# Autodesk Inventor assembly: Ensamble Atril
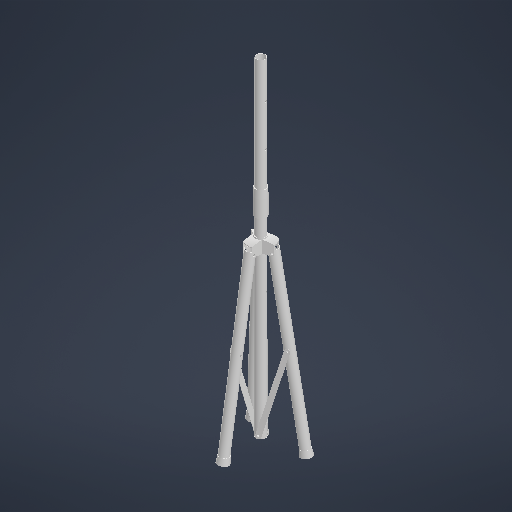
[picture p0: Inventor's stored thumbnail of the model, 512x512]
Saved by Autodesk Inventor 2026.2 (Build 302298000, 298)
## iProperties
Created: 2026-01-05
Part Number: Ensamble Atril
Document SubType Name: Assembly
Designer: vicho
Author: vicho
## Documents named in this file (8)
- C:\Users\vicho\OneDrive\Documentos\PROYECTOS INVENTOR\atril\Ensamble Atril.iam
- C:\Users\vicho\OneDrive\Documentos\PROYECTOS INVENTOR\atril\Pieza37.ipt
- C:\Users\vicho\OneDrive\Documentos\PROYECTOS INVENTOR\atril\Pieza38.ipt
- C:\Users\vicho\OneDrive\Documentos\PROYECTOS INVENTOR\atril\Pieza39.ipt
- C:\Users\vicho\OneDrive\Documentos\PROYECTOS INVENTOR\atril\Pieza40.ipt
- C:\Users\vicho\OneDrive\Documentos\PROYECTOS INVENTOR\atril\Pieza41.ipt
- C:\Users\vicho\OneDrive\Documentos\PROYECTOS INVENTOR\atril\Pieza42.ipt
- C:\Users\vicho\OneDrive\Documentos\PROYECTOS INVENTOR\atril\tapapieza 38.ipt
## Components (11 placed, 7 different names)
1. Pieza37:1 — Coincidencia:1, Coincidencia:2, Coincidencia:19
2. Pieza38:1 — Coincidencia:2, Coincidencia:3, Coincidencia:4, Tangente:7, Coincidencia:12, Tangente:8, Coincidencia:14, Tangente:9, Coincidencia:16, Coincidencia:17, Coincidencia:18
3. Pieza39:1 — Coincidencia:6, Tangente:1, Tangente:2, Coincidencia:13
4. Pieza39:2 — Tangente:5, Coincidencia:10, Tangente:6, Coincidencia:11
5. Pieza39:3 — Coincidencia:9, Tangente:4, Coincidencia:15
6. Pieza40:1 — Coincidencia:11, Tangente:7, Coincidencia:12
7. Pieza40:2 — Coincidencia:13, Tangente:8, Coincidencia:14
8. Pieza40:3 — Coincidencia:15, Tangente:9, Coincidencia:16
9. Pieza41:1 — Coincidencia:4, Coincidencia:6, Tangente:1, Tangente:2, Coincidencia:9, Tangente:4, Tangente:5, Coincidencia:10, Tangente:6, Coincidencia:20
10. Pieza42:1 — Nivelación:1, Nivelación:2, Nivelación:3, Coincidencia:1, Coincidencia:3, Coincidencia:20
11. tapapieza 38:1 — Coincidencia:17, Coincidencia:18, Coincidencia:19
## Relationships (28: Mate 17, Tangent 8, Flush 3)
- Nivelación:1 [Flush]: Pieza42:1
- Nivelación:2 [Flush]: Pieza42:1
- Nivelación:3 [Flush]: Pieza42:1
- Coincidencia:1 [Mate]: Pieza37:1 ↔ Pieza42:1
- Coincidencia:2 [Mate]: Pieza37:1 ↔ Pieza38:1
- Coincidencia:3 [Mate]: Pieza38:1 ↔ Pieza42:1
- Coincidencia:4 [Mate]: Pieza38:1 ↔ Pieza41:1
- Coincidencia:6 [Mate]: Pieza39:1 ↔ Pieza41:1
- Tangente:1: Pieza39:1 ↔ Pieza41:1
- Tangente:2: Pieza39:1 ↔ Pieza41:1
- Coincidencia:9 [Mate]: Pieza39:3 ↔ Pieza41:1
- Tangente:4: Pieza39:3 ↔ Pieza41:1
- Tangente:5: Pieza39:2 ↔ Pieza41:1
- Coincidencia:10 [Mate]: Pieza39:2 ↔ Pieza41:1
- Tangente:6: Pieza39:2 ↔ Pieza41:1
- Coincidencia:11 [Mate]: Pieza39:2 ↔ Pieza40:1
- Tangente:7: Pieza38:1 ↔ Pieza40:1
- Coincidencia:12 [Mate]: Pieza38:1 ↔ Pieza40:1
- Coincidencia:13 [Mate]: Pieza39:1 ↔ Pieza40:2
- Tangente:8: Pieza38:1 ↔ Pieza40:2
- Coincidencia:14 [Mate]: Pieza38:1 ↔ Pieza40:2
- Coincidencia:15 [Mate]: Pieza39:3 ↔ Pieza40:3
- Tangente:9: Pieza38:1 ↔ Pieza40:3
- Coincidencia:16 [Mate]: Pieza38:1 ↔ Pieza40:3
- Coincidencia:17 [Mate]: Pieza38:1 ↔ tapapieza 38:1
- Coincidencia:18 [Mate]: Pieza38:1 ↔ tapapieza 38:1
- Coincidencia:19 [Mate]: Pieza37:1 ↔ tapapieza 38:1
- Coincidencia:20 [Mate] (50 mm): Pieza41:1 ↔ Pieza42:1
